# Autodesk Inventor assembly: Base Assembly
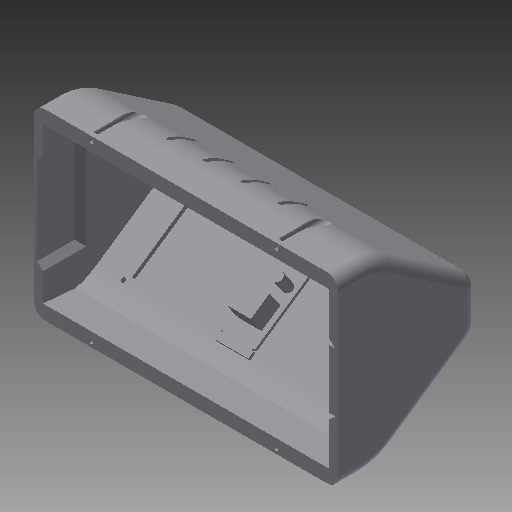
[picture p0: Inventor's stored thumbnail of the model, 512x512]
Saved by Autodesk Inventor 2018 (Build 220112000, 112)
## iProperties
Created: 2019-11-11
Part Number: Base Assembly
Document SubType Name: Assembly
Designer: Jacob
Author: Jacob
## Documents named in this file (6)
- C:\Users\Jacob\git_repos\POE-AIO\CAD Files\New Parts\Base Assembly.iam
- C:\Users\Jacob\git_repos\POE-AIO\CAD Files\More powerful POE Splitter.ipt
- C:\Users\Jacob\git_repos\POE-AIO\CAD Files\New Parts\New Touch Screen Base.ipt
- C:\Users\Jacob\git_repos\POE-AIO\CAD Files\Access Panel.ipt
- C:\Users\Jacob\git_repos\POE-AIO\CAD Files\New Parts\Smaller ethernet holder.ipt
- C:\Users\Jacob\git_repos\POE-AIO\CAD Files\RFID Card Reader.ipt
## Components (5 placed, 5 different names)
1. More powerful POE Splitter:1
2. New Touch Screen Base:1
3. Access Panel:1
4. Smaller ethernet holder:1
5. RFID Card Reader:1
## Relationships (11: Mate 10, Flush 1)
- [Mate]: New Touch Screen Base:1 ↔ Access Panel:1
- [Mate]: New Touch Screen Base:1 ↔ Access Panel:1
- [Mate]: New Touch Screen Base:1 ↔ Access Panel:1
- [Mate]: More powerful POE Splitter:1 ↔ New Touch Screen Base:1
- [Mate]: More powerful POE Splitter:1 ↔ New Touch Screen Base:1
- [Mate]: More powerful POE Splitter:1 ↔ New Touch Screen Base:1
- [Mate]: More powerful POE Splitter:1 ↔ Smaller ethernet holder:1
- [Mate]: More powerful POE Splitter:1 ↔ Smaller ethernet holder:1
- [Flush]: New Touch Screen Base:1 ↔ RFID Card Reader:1
- [Mate]: New Touch Screen Base:1 ↔ RFID Card Reader:1
- [Mate]: New Touch Screen Base:1 ↔ RFID Card Reader:1
